# Autodesk Inventor assembly: supports
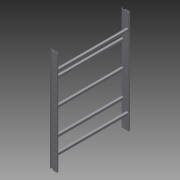
[picture p0: Inventor's stored thumbnail of the model, 180x180]
Saved by Autodesk Inventor 2013 (Build 170138000, 138)
## iProperties
Created: 2012-10-21
Part Number: supports
Document SubType Name: Weldment
Designer: Istvan
Weld Material: Welded Aluminum-6061
Mass: 4701.04 g
Surface Area: 39626.7 cm^2
Volume: 4701.04 cm^3
Density: 1 g/cm^3
Author: Istvan
## Documents named in this file (7)
- C:\Users\istvan.burbank\Documents\GitHub\Crown-Fire\CAD\Frame\Supports\supports.iam
- D:\GitHub\Crown-Fire\CAD\Templates\squareTube_1.5.ipt
- C:\Users\istvan.burbank\Documents\GitHub\Crown-Fire\CAD\Frame\Supports\tableBrace-l.ipt
- C:\Users\istvan.burbank\Documents\GitHub\Crown-Fire\CAD\Frame\Supports\frameBottomChannel.ipt
- E:\GitHub\Crown-Fire\CAD\Templates\cChannel2x1.ipt
- C:\Users\istvan.burbank\Documents\GitHub\Crown-Fire\CAD\Frame\Supports\sideRail.ipt
- E:\GitHub\Crown-Fire\CAD\Templates\squareTube_1x2.ipt
## Components (9 placed, 3 different names)
1. sideRail:1 — Mate:20, Flush:25, Flush:26, Mate:21, Flush:29, Mate:24, Flush:33, Flush:34, Flush:37, Flush:38
2. tableBrace-l:4 — Mate:22, Flush:30, Mate:24, Flush:33, Flush:34, Mate:29
3. tableBrace-l:14 — Mate:20, Flush:25, Flush:26, Mate:28
4. frameBottomChannel:1 — Mate:21, Flush:37, Flush:38, Flush:39, Flush:40, Flush:41
5. frameBottomChannel:2 — Mate:23, Flush:35, Flush:36, Mate:25, Mate:26, Mate:27
6. sideRail:2 — Mate:22, Flush:29, Flush:30, Mate:23, Flush:35, Flush:36
7. tableBrace-l:15 — Mate:26, Flush:40, Mate:30
8. tableBrace-l:16 — Mate:27, Flush:41, Mate:28, Mate:30
9. tableBrace-l:17 — Mate:25, Flush:39, Mate:29
## Relationships (24: Flush 13, Mate 11)
- Mate:20: sideRail:1 ↔ tableBrace-l:14
- Flush:25 (-254 mm): sideRail:1 ↔ tableBrace-l:14
- Flush:26: sideRail:1 ↔ tableBrace-l:14
- Mate:21: sideRail:1 ↔ frameBottomChannel:1
- Mate:22: tableBrace-l:4 ↔ sideRail:2
- Flush:29: sideRail:1 ↔ sideRail:2
- Flush:30: tableBrace-l:4 ↔ sideRail:2
- Mate:23: frameBottomChannel:2 ↔ sideRail:2
- Mate:24: sideRail:1 ↔ tableBrace-l:4
- Flush:33: sideRail:1 ↔ tableBrace-l:4
- Flush:34 (254 mm): sideRail:1 ↔ tableBrace-l:4
- Flush:35: frameBottomChannel:2 ↔ sideRail:2
- Flush:36: frameBottomChannel:2 ↔ sideRail:2
- Flush:37: sideRail:1 ↔ frameBottomChannel:1
- Flush:38: sideRail:1 ↔ frameBottomChannel:1
- Mate:25: frameBottomChannel:2 ↔ tableBrace-l:17
- Mate:26: frameBottomChannel:2 ↔ tableBrace-l:15
- Mate:27: frameBottomChannel:2 ↔ tableBrace-l:16
- Flush:39: frameBottomChannel:1 ↔ tableBrace-l:17
- Flush:40: frameBottomChannel:1 ↔ tableBrace-l:15
- Flush:41: frameBottomChannel:1 ↔ tableBrace-l:16
- Mate:28 (152.4 mm): tableBrace-l:14 ↔ tableBrace-l:16
- Mate:29 (152.4 mm): tableBrace-l:4 ↔ tableBrace-l:17
- Mate:30 (412.75 mm): tableBrace-l:15 ↔ tableBrace-l:16
